# Autodesk Inventor assembly: Assembly_fnal
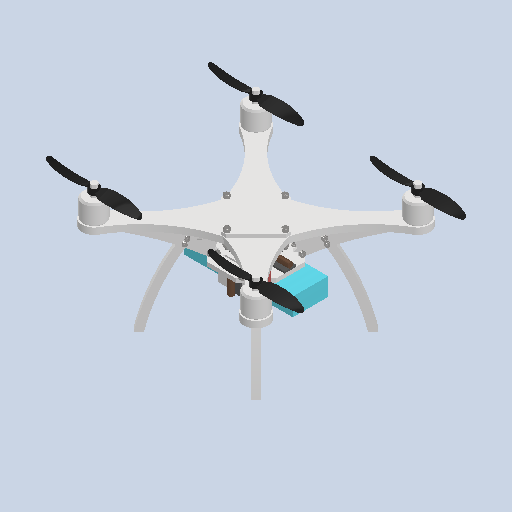
[picture p0: Inventor's stored thumbnail of the model, 512x512]
Saved by Autodesk Inventor 2025.2 (Build 292293000, 293)
## iProperties
Created: 2025-04-05
Part Number: Assembly_fnal
Document SubType Name: Assembly
Designer: mirewn
Author: mirewn
## Documents named in this file (21)
- C:\Users\mirewn\OneDrive - Universitatea Politehnica Bucuresti\AA- Projects\Drona\v4\Assembly.iam
- C:\Users\mirewn\OneDrive - Universitatea Politehnica Bucuresti\AA- Projects\Drona\v4\bottom.ipt
- C:\Users\mirewn\OneDrive - Universitatea Politehnica Bucuresti\AA- Projects\Drona\v4\arm.ipt
- C:\Users\mirewn\OneDrive - Universitatea Politehnica Bucuresti\AA- Projects\Drona\v4\Eletronics\Antenne.ipt
- C:\Users\mirewn\OneDrive - Universitatea Politehnica Bucuresti\AA- Projects\Drona\v4\Eletronics\FC.ipt
- C:\Users\mirewn\OneDrive - Universitatea Politehnica Bucuresti\AA- Projects\Drona\v4\Eletronics\phat ahh battery.ipt
- C:\Users\mirewn\OneDrive - Universitatea Politehnica Bucuresti\AA- Projects\Drona\v4\leg.ipt
- C:\Users\mirewn\OneDrive - Universitatea Politehnica Bucuresti\AA- Projects\Drona\v4\Eletronics\Telemetrie.ipt
- C:\Users\mirewn\OneDrive - Universitatea Politehnica Bucuresti\AA- Projects\Drona\v4\top.ipt
- C:\Users\mirewn\OneDrive - Universitatea Politehnica Bucuresti\AA- Projects\rizzler time\motor.ipt
- C:\Users\mirewn\OneDrive - Universitatea Politehnica Bucuresti\AA- Projects\Drona\v4\Eletronics\Propeller.ipt
- C:\Users\mirewn\OneDrive - Universitatea Politehnica Bucuresti\AA- Projects\Drona\v4\hook.ipt
- C:\Users\mirewn\OneDrive - Universitatea Politehnica Bucuresti\AA- Projects\Drona\v4\hook_arm.ipt
- C:\Users\mirewn\OneDrive - Universitatea Politehnica Bucuresti\AA- Projects\Drona\v4\Eletronics\Laser.ipt
- C:\Users\mirewn\Documents\Inventor\Content Center Files\R2025\en-US\DIN 912\DIN 912 - M3 x 0.5 x 25 x 18.ipt
- C:\Users\mirewn\Documents\Inventor\Content Center Files\R2025\en-US\DIN 912\DIN 912 - M3 x 0.5 x 12 x 10.75.ipt
- C:\Users\mirewn\Documents\Inventor\Content Center Files\R2025\en-US\DIN 985\DIN 985 - M3.ipt
- C:\Users\mirewn\Documents\Inventor\Content Center Files\R2025\en-US\DIN 985\DIN 985 - M4.ipt
- C:\Users\mirewn\Documents\Inventor\Content Center Files\R2025\en-US\DIN 912\DIN 912 - M4 x 0.7 x 20 x 18.25.ipt
- C:\Users\mirewn\Documents\Inventor\Content Center Files\R2025\en-US\DIN 912\DIN 912 - M3 x 0.5 x 16 x 14.75.ipt
- C:\Users\mirewn\OneDrive - Universitatea Politehnica Bucuresti\AA- Projects\Drona\v4\Eletronics\Antenne2.ipt
## Components (70 placed, 20 different names)
1. bottom:1 — Mate:1, Mate:2, Mate:3, Mate:6, Mate:7, Mate:8, Mate:9, Flush:2, Flush:3, Mate:13, Flush:4, Mate:14, Mate:24, Mate:25, Mate:26, Mate:29, Flush:5, Mate:30, Insert:20, Insert:21, Insert:22, Insert:23, Mate:35, Mate:36, Mate:37, Mate:38
2. Antenne:1 — Mate:4, Mate:5, Flush:1
3. FC:1 — Mate:6, Mate:7, Mate:8
4. phat ahh battery:1 — Mate:9, Flush:2, Flush:3
5. Telemetrie:1 — Mate:13, Flush:4, Mate:14
6. top:1 — Mate:15, Mate:17, Mate:18, Insert:9, Insert:10, Insert:11, Insert:12
7. hook:1 — Mate:24, Mate:25, Mate:26, Mate:27, Mate:28, Mate:31, Flush:6, Mate:32, Insert:4, Insert:5, Insert:6, Insert:7, Insert:8, Insert:24, Mate:42, Mate:43
8. hook_arm:1 — Mate:27, Mate:28, Mate:35, Mate:36, Mate:37, Mate:38, Mate:39, Mate:40, Mate:41, Flush:9, Flush:10, Mate:42, Mate:43, Mate:44, Mate:45
9. Laser:1 — Mate:29, Flush:5, Mate:30
10. Laser:2 — Mate:31, Flush:6, Mate:32, Mate:41, Flush:9, Flush:10
11. DIN 912 - replaced by DIN EN ISO 4762 M3 x 12:2 — Insert:4, Mate:39
12. DIN 912 - replaced by DIN EN ISO 4762 M3 x 12:5 — Insert:5
13. DIN 912 - replaced by DIN EN ISO 4762 M3 x 12:4 — Insert:6, Mate:40
14. DIN 912 - replaced by DIN EN ISO 4762 M3 x 12:3 — Insert:7
15. DIN 912 - replaced by DIN EN ISO 4762 M3 x 16:1 — Insert:8, Mate:44
16. DIN 912 - replaced by DIN EN ISO 4762 M4 x 20:4 — Insert:9
17. DIN 912 - replaced by DIN EN ISO 4762 M4 x 20:3 — Insert:10
18. DIN 912 - replaced by DIN EN ISO 4762 M4 x 20:2 — Insert:11
19. DIN 912 - replaced by DIN EN ISO 4762 M4 x 20:1 — Insert:12
20. DIN 985 - replaced by DIN EN ISO 10511 M4:1 — Insert:16
21. DIN 985 - replaced by DIN EN ISO 10511 M4:2 — Insert:17
22. DIN 985 - replaced by DIN EN ISO 10511 M4:3 — Insert:18
23. DIN 985 - replaced by DIN EN ISO 10511 M4:4 — Insert:19
24. DIN 985 - replaced by DIN EN ISO 10511 M3:4 — Insert:20
25. DIN 985 - replaced by DIN EN ISO 10511 M3:5 — Insert:21
26. DIN 985 - replaced by DIN EN ISO 10511 M3:6 — Insert:22
27. DIN 985 - replaced by DIN EN ISO 10511 M3:7 — Insert:23
28. DIN 985 - replaced by DIN EN ISO 10511 M3:8 — Insert:24, Mate:45
29. Antenne2:1 — Flush:7, Mate:33
30. Antenne2:2 — Flush:8, Mate:34
31. arm:1 — Mate:1, Mate:2, Mate:3, Mate:5, Flush:1, Insert:1, Insert:2, Insert:3, Insert:13, Insert:14, Insert:15, Insert:19
32. arm:2 — Mate:10, Mate:11, Mate:12, Mate:15, Insert:16
33. arm:3 — Mate:17, Mate:19, Mate:20, Mate:21, Insert:17, Flush:8, Mate:34
34. arm:4 — Mate:4, Mate:18, Insert:18, Flush:7, Mate:33
35. leg:1 — Mate:10, Mate:11, Mate:12
36. leg:2
37. leg:3
38. leg:4
39. motor:1 — Mate:19, Mate:20, Mate:21, Mate:22, Mate:23
40. Propeller:1 — Mate:22, Mate:23
41. motor:2
42. Propeller:2
43. motor:3
44. Propeller:3
45. motor:4
46. Propeller:4
47. DIN 985 - replaced by DIN EN ISO 10511 M3:2 — Insert:14
48. DIN 912 - replaced by DIN EN ISO 4762 M3 x 25:1 — Insert:1
49. DIN 912 - replaced by DIN EN ISO 4762 M3 x 25:2 — Insert:2
50. DIN 985 - replaced by DIN EN ISO 10511 M3:1 — Insert:13
51. DIN 985 - replaced by DIN EN ISO 10511 M3:3 — Insert:15
52. DIN 912 - replaced by DIN EN ISO 4762 M3 x 25:3 — Insert:3
53. DIN 985 - replaced by DIN EN ISO 10511 M3:9
54. DIN 912 - replaced by DIN EN ISO 4762 M3 x 25:4
55. DIN 912 - replaced by DIN EN ISO 4762 M3 x 25:5
56. DIN 985 - replaced by DIN EN ISO 10511 M3:10
57. DIN 985 - replaced by DIN EN ISO 10511 M3:11
58. DIN 912 - replaced by DIN EN ISO 4762 M3 x 25:6
59. DIN 985 - replaced by DIN EN ISO 10511 M3:12
60. DIN 912 - replaced by DIN EN ISO 4762 M3 x 25:7
61. DIN 912 - replaced by DIN EN ISO 4762 M3 x 25:8
62. DIN 985 - replaced by DIN EN ISO 10511 M3:13
63. DIN 985 - replaced by DIN EN ISO 10511 M3:14
64. DIN 912 - replaced by DIN EN ISO 4762 M3 x 25:9
65. DIN 985 - replaced by DIN EN ISO 10511 M3:15
66. DIN 912 - replaced by DIN EN ISO 4762 M3 x 25:10
67. DIN 912 - replaced by DIN EN ISO 4762 M3 x 25:11
68. DIN 985 - replaced by DIN EN ISO 10511 M3:16
69. DIN 985 - replaced by DIN EN ISO 10511 M3:17
70. DIN 912 - replaced by DIN EN ISO 4762 M3 x 25:12
## Component patterns: (4 elements, first: arm:1), (4 elements, first: leg:1), (4 elements, first: motor:1 + Propeller:1), (4 elements, first: DIN 985 - replaced by DIN EN ISO 10511 M3:2 + DIN 912 - replaced by DIN EN ISO 4762 M3 x 25:1 + DIN 912 - replaced by DIN EN ISO 4762 M3 x 25:2 + DIN 985 - replaced by DIN EN ISO 10511 M3:1 + DIN 985 - replaced by DIN EN ISO 10511 M3:3 + DIN 912 - replaced by DIN EN ISO 4762 M3 x 25:3)
## Relationships (78: Mate 44, Insert 24, Flush 10)
- Mate:1 (0.3 mm): bottom:1 ↔ arm:1
- Mate:2: bottom:1 ↔ arm:1
- Mate:3 (0.25 mm): bottom:1 ↔ arm:1
- Mate:4 (2 mm): Antenne:1 ↔ arm:4
- Mate:5 (10 mm): Antenne:1 ↔ arm:1
- Flush:1 (-2 mm): Antenne:1 ↔ arm:1
- Mate:6: bottom:1 ↔ FC:1
- Mate:7: bottom:1 ↔ FC:1
- Mate:8: bottom:1 ↔ FC:1
- Mate:9: bottom:1 ↔ phat ahh battery:1
- Flush:2 (21 mm): bottom:1 ↔ phat ahh battery:1
- Flush:3 (25 mm): bottom:1 ↔ phat ahh battery:1
- Mate:10: arm:2 ↔ leg:1
- Mate:11: arm:2 ↔ leg:1
- Mate:12 (0.25 mm): arm:2 ↔ leg:1
- Mate:13: bottom:1 ↔ Telemetrie:1
- Flush:4 (5 mm): bottom:1 ↔ Telemetrie:1
- Mate:14 (4 mm): bottom:1 ↔ Telemetrie:1
- Mate:15: top:1 ↔ arm:2
- Mate:17: top:1 ↔ arm:3
- Mate:18: top:1 ↔ arm:4
- Mate:19: arm:3 ↔ motor:1
- Mate:20: arm:3 ↔ motor:1
- Mate:21: arm:3 ↔ motor:1
- Mate:22: motor:1 ↔ Propeller:1
- Mate:23 (4 mm): motor:1 ↔ Propeller:1
- Mate:24: bottom:1 ↔ hook:1
- Mate:25: bottom:1 ↔ hook:1
- Mate:26: bottom:1 ↔ hook:1
- Mate:27: hook:1 ↔ hook_arm:1
- Mate:28 (0.1 mm): hook:1 ↔ hook_arm:1
- Mate:29: bottom:1 ↔ Laser:1
- Flush:5: bottom:1 ↔ Laser:1
- Mate:30 (10.31 mm): bottom:1 ↔ Laser:1
- Mate:31: hook:1 ↔ Laser:2
- Flush:6 (2 mm): hook:1 ↔ Laser:2
- Mate:32 (14.5 mm): hook:1 ↔ Laser:2
- Insert:1: arm:1 ↔ DIN 912 - replaced by DIN EN ISO 4762 M3 x 25:1
- Insert:2: arm:1 ↔ DIN 912 - replaced by DIN EN ISO 4762 M3 x 25:2
- Insert:3: arm:1 ↔ DIN 912 - replaced by DIN EN ISO 4762 M3 x 25:3
- Insert:4: hook:1 ↔ DIN 912 - replaced by DIN EN ISO 4762 M3 x 12:2
- Insert:5: hook:1 ↔ DIN 912 - replaced by DIN EN ISO 4762 M3 x 12:5
- Insert:6: hook:1 ↔ DIN 912 - replaced by DIN EN ISO 4762 M3 x 12:4
- Insert:7: hook:1 ↔ DIN 912 - replaced by DIN EN ISO 4762 M3 x 12:3
- Insert:8: hook:1 ↔ DIN 912 - replaced by DIN EN ISO 4762 M3 x 16:1
- Insert:9: top:1 ↔ DIN 912 - replaced by DIN EN ISO 4762 M4 x 20:4
- Insert:10: top:1 ↔ DIN 912 - replaced by DIN EN ISO 4762 M4 x 20:3
- Insert:11: top:1 ↔ DIN 912 - replaced by DIN EN ISO 4762 M4 x 20:2
- Insert:12: top:1 ↔ DIN 912 - replaced by DIN EN ISO 4762 M4 x 20:1
- Insert:13: arm:1 ↔ DIN 985 - replaced by DIN EN ISO 10511 M3:1
- Insert:14: arm:1 ↔ DIN 985 - replaced by DIN EN ISO 10511 M3:2
- Insert:15: arm:1 ↔ DIN 985 - replaced by DIN EN ISO 10511 M3:3
- Insert:16: DIN 985 - replaced by DIN EN ISO 10511 M4:1 ↔ arm:2
- Insert:17: DIN 985 - replaced by DIN EN ISO 10511 M4:2 ↔ arm:3
- Insert:18: DIN 985 - replaced by DIN EN ISO 10511 M4:3 ↔ arm:4
- Insert:19: DIN 985 - replaced by DIN EN ISO 10511 M4:4 ↔ arm:1
- Insert:20: bottom:1 ↔ DIN 985 - replaced by DIN EN ISO 10511 M3:4
- Insert:21: bottom:1 ↔ DIN 985 - replaced by DIN EN ISO 10511 M3:5
- Insert:22: bottom:1 ↔ DIN 985 - replaced by DIN EN ISO 10511 M3:6
- Insert:23: bottom:1 ↔ DIN 985 - replaced by DIN EN ISO 10511 M3:7
- Insert:24: hook:1 ↔ DIN 985 - replaced by DIN EN ISO 10511 M3:8
- Flush:7 (-3 mm): Antenne2:1 ↔ arm:4
- Mate:33: Antenne2:1 ↔ arm:4
- Flush:8 (-3 mm): Antenne2:2 ↔ arm:3
- Mate:34: Antenne2:2 ↔ arm:3
- Mate:35: bottom:1 ↔ hook_arm:1
- Mate:36: bottom:1 ↔ hook_arm:1
- Mate:37: bottom:1 ↔ hook_arm:1
- Mate:38: bottom:1 ↔ hook_arm:1
- Mate:39: hook_arm:1 ↔ DIN 912 - replaced by DIN EN ISO 4762 M3 x 12:2
- Mate:40: hook_arm:1 ↔ DIN 912 - replaced by DIN EN ISO 4762 M3 x 12:4
- Mate:41: hook_arm:1 ↔ Laser:2
- Flush:9: hook_arm:1 ↔ Laser:2
- Flush:10 (14 mm): hook_arm:1 ↔ Laser:2
- Mate:42: hook:1 ↔ hook_arm:1
- Mate:43 (0.1 mm): hook:1 ↔ hook_arm:1
- Mate:44: hook_arm:1 ↔ DIN 912 - replaced by DIN EN ISO 4762 M3 x 16:1
- Mate:45: hook_arm:1 ↔ DIN 985 - replaced by DIN EN ISO 10511 M3:8
